# Autodesk Inventor assembly: BAO Sign
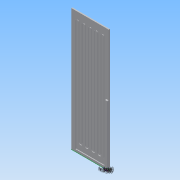
[picture p0: Inventor's stored thumbnail of the model, 180x180]
Saved by Autodesk Inventor 2013 (Build 170138000, 138)
## iProperties
Created: 2018-07-18
Part Number: BAO Sign
Document SubType Name: Assembly
Designer: Jeff Vyduna
Author: Jeff Vyduna
## Documents named in this file (5)
- \\vmware-host\Shared Folders\Desktop\Hot fresh bao sign\CAD\BAO Sign.iam
- \\vmware-host\Shared Folders\Desktop\Hot fresh bao sign\CAD\Sign ply back, v3 separate parts.ipt
- \\vmware-host\Shared Folders\Desktop\Hot fresh bao sign\CAD\Sideborder.ipt
- \\vmware-host\Shared Folders\Desktop\Hot fresh bao sign\CAD\SideborderInverse.ipt
- \\vmware-host\Shared Folders\Desktop\Hot fresh bao sign\CAD\TopBottomBorder.ipt
## Components (6 placed, 4 different names)
1. Sign ply back, v3 separate parts:1 — Flush:1, Flush:2, Flush:3, Mate:1, Flush:4, Flush:5, Flush:6, Mate:2, Flush:7, Mate:3, Flush:8, Flush:9, Flush:10
2. Sideborder:1 — Flush:1, Flush:2
3. SideborderInverse:1 — Flush:3, Mate:1, Flush:4
4. Sideborder:2 — Flush:5, Flush:6, Mate:2
5. SideborderInverse:2 — Flush:7, Mate:3, Flush:8
6. TopBottomBorder:1 — Flush:9, Flush:10
## Relationships (13: Flush 10, Mate 3)
- Flush:1: Sign ply back, v3 separate parts:1 ↔ Sideborder:1
- Flush:2: Sign ply back, v3 separate parts:1 ↔ Sideborder:1
- Flush:3: Sign ply back, v3 separate parts:1 ↔ SideborderInverse:1
- Mate:1: Sign ply back, v3 separate parts:1 ↔ SideborderInverse:1
- Flush:4: Sign ply back, v3 separate parts:1 ↔ SideborderInverse:1
- Flush:5: Sign ply back, v3 separate parts:1 ↔ Sideborder:2
- Flush:6: Sign ply back, v3 separate parts:1 ↔ Sideborder:2
- Mate:2: Sign ply back, v3 separate parts:1 ↔ Sideborder:2
- Flush:7: Sign ply back, v3 separate parts:1 ↔ SideborderInverse:2
- Mate:3: Sign ply back, v3 separate parts:1 ↔ SideborderInverse:2
- Flush:8: Sign ply back, v3 separate parts:1 ↔ SideborderInverse:2
- Flush:9: Sign ply back, v3 separate parts:1 ↔ TopBottomBorder:1
- Flush:10: Sign ply back, v3 separate parts:1 ↔ TopBottomBorder:1
## Named parameters: signW = 609.6 mm, borderLap = 12.7 mm, borderW = 38.1 mm, borderH = 25.4 mm, velcroH = 2.54 mm, panelH = 5.1308 mm, panelHClear = 0.79375 mm, signH = 1981.2 mm
